# Autodesk Inventor assembly: Муфта в сборе
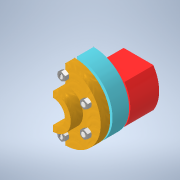
[picture p0: Inventor's stored thumbnail of the model, 180x180]
Saved by Autodesk Inventor 2021 (Build 250183000, 183)
## iProperties
Created: 2023-04-15
Part Number: Муфта в сборе
Document SubType Name: Assembly
Designer: gdevc
Author: gdevc
## Documents named in this file (11)
- C:\Users\gdevc\OneDrive\Рабочий стол\Курсач\DetaliMashine\Новая папка\Муфта в сборе.iam
- C:\Users\gdevc\OneDrive\Рабочий стол\Курсач\DetaliMashine\Новая папка\Муфта_Корпус.ipt
- C:\Users\gdevc\OneDrive\Рабочий стол\Курсач\DetaliMashine\Новая папка\Палец_ребрышко.ipt
- C:\Users\gdevc\OneDrive\Рабочий стол\Курсач\DetaliMashine\Новая папка\ANSI B 18.2.4.1 M - M10 x 1,5Style 1.ipt
- C:\Users\gdevc\OneDrive\Рабочий стол\Курсач\DetaliMashine\Новая папка\Демфер пальца.ipt
- C:\Users\gdevc\OneDrive\Рабочий стол\Курсач\DetaliMashine\Новая папка\Проставка.ipt
- C:\Users\gdevc\OneDrive\Рабочий стол\Курсач\DetaliMashine\Новая папка\Винт A.M10-6gx18 ГОСТ 17473-80.ipt
- C:\Users\gdevc\OneDrive\Рабочий стол\Курсач\DetaliMashine\Новая папка\Штрифт.ipt
- C:\Users\gdevc\OneDrive\Рабочий стол\Курсач\DetaliMashine\Новая папка\Втулка_Штрифта.ipt
- C:\Users\gdevc\OneDrive\Рабочий стол\Курсач\DetaliMashine\Новая папка\Втулка_Штрифта_MIR.ipt
- C:\Users\gdevc\OneDrive\Рабочий стол\Курсач\DetaliMashine\Новая папка\Скольжение.ipt
## Components (30 placed, 10 different names)
1. Муфта_Корпус:1 — Совмещение:1, Совмещение:2, Совмещение:4, Совмещение:9, Совмещение:10, Совмещение:11, Совмещение:13, Заподлицо:1
2. Винт A.M10-6gx18 ГОСТ 17473-80:1 — Совмещение:9, Совмещение:10, Угол:3
3. Штрифт:1 — Совмещение:11, Совмещение:12
4. Втулка_Штрифта:1 — Совмещение:12
5. Втулка_Штрифта_MIR:1
6. Скольжение:1 — Совмещение:13, Заподлицо:1
7. Демфер пальца:1 — Совмещение:5, Совмещение:6, Совмещение:7, Совмещение:8
8. Палец_ребрышко:1 — Совмещение:1, Совмещение:2, Совмещение:3, Угол:1, Совмещение:5, Совмещение:6
9. ANSI B 18.2.4.1 M - M10 x 1,5Style 1:1 — Совмещение:3, Угол:1, Угол:2, Совмещение:4
10. Демфер пальца:2
11. Палец_ребрышко:2
12. ANSI B 18.2.4.1 M - M10 x 1,5Style 1:2
13. Демфер пальца:3
14. Палец_ребрышко:3
15. ANSI B 18.2.4.1 M - M10 x 1,5Style 1:3
16. Демфер пальца:4
17. Палец_ребрышко:4
18. ANSI B 18.2.4.1 M - M10 x 1,5Style 1:4
19. Демфер пальца:5
20. Палец_ребрышко:5
21. ANSI B 18.2.4.1 M - M10 x 1,5Style 1:5
22. Демфер пальца:6
23. Палец_ребрышко:6
24. ANSI B 18.2.4.1 M - M10 x 1,5Style 1:6
25. Проставка:1 — Совмещение:7, Совмещение:8
26. Проставка:2
27. Проставка:3
28. Проставка:4
29. Проставка:5
30. Проставка:6
## Component patterns: (6 elements, first: Демфер пальца:1 + Палец_ребрышко:1 + ANSI B 18.2.4.1 M - M10 x 1,5Style 1:1), (6 elements, first: Проставка:1)
## Relationships (17: Mate 13, Angle 3, Flush 1)
- Совмещение:1 [Mate]: Муфта_Корпус:1 ↔ Палец_ребрышко:1
- Совмещение:2 [Mate]: Муфта_Корпус:1 ↔ Палец_ребрышко:1
- Совмещение:3 [Mate]: Палец_ребрышко:1 ↔ ANSI B 18.2.4.1 M - M10 x 1,5Style 1:1
- Угол:1 [Angle] (0 deg): Палец_ребрышко:1 ↔ ANSI B 18.2.4.1 M - M10 x 1,5Style 1:1
- Угол:2 [Angle] (0 deg): ANSI B 18.2.4.1 M - M10 x 1,5Style 1:1
- Совмещение:4 [Mate]: Муфта_Корпус:1 ↔ ANSI B 18.2.4.1 M - M10 x 1,5Style 1:1
- Совмещение:5 [Mate]: Демфер пальца:1 ↔ Палец_ребрышко:1
- Совмещение:6 [Mate]: Демфер пальца:1 ↔ Палец_ребрышко:1
- Совмещение:7 [Mate]: Демфер пальца:1 ↔ Проставка:1
- Совмещение:8 [Mate]: Демфер пальца:1 ↔ Проставка:1
- Совмещение:9 [Mate]: Муфта_Корпус:1 ↔ Винт A.M10-6gx18 ГОСТ 17473-80:1
- Совмещение:10 [Mate]: Муфта_Корпус:1 ↔ Винт A.M10-6gx18 ГОСТ 17473-80:1
- Совмещение:11 [Mate]: Муфта_Корпус:1 ↔ Штрифт:1
- Совмещение:12 [Mate]: Штрифт:1 ↔ Втулка_Штрифта:1
- Угол:3 [Angle] (0 deg): Винт A.M10-6gx18 ГОСТ 17473-80:1
- Совмещение:13 [Mate]: Муфта_Корпус:1 ↔ Скольжение:1
- Заподлицо:1 [Flush]: Муфта_Корпус:1 ↔ Скольжение:1
